# Autodesk Inventor assembly: jet done model
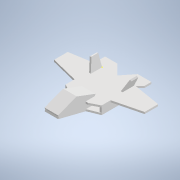
[picture p0: Inventor's stored thumbnail of the model, 180x180]
Saved by Autodesk Inventor 2020 (Build 240168000, 168)
## iProperties
Created: 2019-05-16
Part Number: jet done model
Document SubType Name: Assembly
Designer: kangh
Author: kangh
## Documents named in this file (8)
- C:\Users\kangh\Desktop\Project\cad\jet done model.iam
- C:\Users\kangh\Desktop\Project\cad\main body jet.ipt
- C:\Users\kangh\Desktop\Project\cad\side wing jet.ipt
- C:\Users\kangh\Desktop\Project\cad\sidewing 2 jet.ipt
- C:\Users\kangh\Desktop\Project\cad\side bottom jet.ipt
- C:\Users\kangh\Desktop\Project\cad\head bottom jet.ipt
- C:\Users\kangh\Desktop\Project\cad\head top jet.ipt
- C:\Users\kangh\Desktop\Project\cad\head side jet.ipt
## Components (9 placed, 7 different names)
1. main body jet:1 — Mate:9, Flush:8, Mate:10, Mate:11
2. side wing jet:1 — Mate:11
3. sidewing 2 jet:1 — Mate:10
4. side bottom jet:1 — Mate:2, Flush:3, Flush:4
5. side bottom jet:2 — Mate:1, Flush:1, Flush:2, Flush:8
6. head bottom jet:1 — Mate:1, Flush:1, Flush:2, Mate:2, Flush:3, Flush:4, Mate:3, Mate:4, Flush:5, Mate:5, Mate:6, Flush:6
7. head top jet:1 — Mate:7, Flush:7, Mate:8
8. head side jet:1 — Mate:3, Mate:4, Flush:5, Mate:7
9. head side jet:2 — Mate:5, Mate:6, Flush:6, Flush:7, Mate:8, Mate:9
## Relationships (19: Mate 11, Flush 8)
- Mate:1: side bottom jet:2 ↔ head bottom jet:1
- Flush:1: side bottom jet:2 ↔ head bottom jet:1
- Flush:2: side bottom jet:2 ↔ head bottom jet:1
- Mate:2: side bottom jet:1 ↔ head bottom jet:1
- Flush:3: side bottom jet:1 ↔ head bottom jet:1
- Flush:4: side bottom jet:1 ↔ head bottom jet:1
- Mate:3: head bottom jet:1 ↔ head side jet:1
- Mate:4: head bottom jet:1 ↔ head side jet:1
- Flush:5: head bottom jet:1 ↔ head side jet:1
- Mate:5: head bottom jet:1 ↔ head side jet:2
- Mate:6: head bottom jet:1 ↔ head side jet:2
- Flush:6: head bottom jet:1 ↔ head side jet:2
- Mate:7: head top jet:1 ↔ head side jet:1
- Flush:7: head top jet:1 ↔ head side jet:2
- Mate:8: head top jet:1 ↔ head side jet:2
- Mate:9: main body jet:1 ↔ head side jet:2
- Flush:8: main body jet:1 ↔ side bottom jet:2
- Mate:10: main body jet:1 ↔ sidewing 2 jet:1
- Mate:11: main body jet:1 ↔ side wing jet:1
